# Autodesk Inventor assembly: Full Assembly
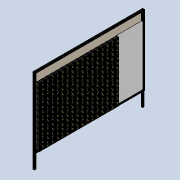
[picture p0: Inventor's stored thumbnail of the model, 180x180]
Saved by Autodesk Inventor 2022 (Build 260153000, 153)
## iProperties
Created: 2023-02-26
Part Number: Full Assembly
Document SubType Name: Assembly
Designer: byrne
Author: byrne
## Documents named in this file (7)
- C:\Users\byrne\OneDrive\Documents\Inventor\RAI\Full Assembly.iam
- C:\Users\byrne\OneDrive\Documents\Inventor\RAI\Backboard.ipt
- C:\Users\byrne\OneDrive\Documents\Inventor\RAI\56in T-Extrusion.ipt
- C:\Users\byrne\OneDrive\Documents\Inventor\RAI\70in T-Extrusion.ipt
- C:\Users\byrne\OneDrive\Documents\Inventor\RAI\Unit.iam
- C:\Users\byrne\OneDrive\Documents\Inventor\RAI\Sponsor and Ad Panel.ipt
- C:\Users\byrne\OneDrive\Documents\Inventor\RAI\98164A450_316 Stainless Steel Button Head Hex Drive Screw.ipt
## Components (202 placed, 6 different names)
1. Sponsor and Ad Panel:1 — Mate:9, Flush:11, Mate:10, Insert:1, Insert:2, Insert:3, Insert:4
2. 98164A450_316 Stainless Steel Button Head Hex Drive Screw:1 — Insert:3
3. 98164A450_316 Stainless Steel Button Head Hex Drive Screw:2 — Insert:2
4. 98164A450_316 Stainless Steel Button Head Hex Drive Screw:3 — Insert:1
5. 98164A450_316 Stainless Steel Button Head Hex Drive Screw:4 — Insert:4
6. Backboard:1 — Flush:1, Mate:1, Flush:2, Flush:4, Mate:2, Flush:5, Flush:7, Mate:3, Flush:8, Mate:6, Mate:7, Flush:10, Mate:10, Flush:12
7. 56in T-Extrusion:1 — Flush:4, Mate:2, Flush:5, Mate:8
8. 70in T-Extrusion:1 — Flush:8, Mate:6, Mate:8
9. 56in T-Extrusion:2 — Flush:1, Mate:1, Flush:2, Mate:4
10. 70in T-Extrusion:2 — Flush:7, Mate:3, Mate:4
11. Unit:1 [sub-assembly] — Mate:7, Flush:10
12. Unit:2 [sub-assembly]
13. Unit:3 [sub-assembly]
14. Unit:4 [sub-assembly]
15. Unit:5 [sub-assembly]
16. Unit:6 [sub-assembly]
17. Unit:7 [sub-assembly]
18. Unit:8 [sub-assembly]
19. Unit:9 [sub-assembly]
20. Unit:10 [sub-assembly]
21. Unit:11 [sub-assembly]
22. Unit:12 [sub-assembly]
23. Unit:13 [sub-assembly]
24. Unit:14 [sub-assembly]
25. Unit:15 [sub-assembly]
26. Unit:16 [sub-assembly]
27. Unit:17 [sub-assembly]
28. Unit:18 [sub-assembly]
29. Unit:19 [sub-assembly]
30. Unit:20 [sub-assembly]
31. Unit:21 [sub-assembly]
32. Unit:22 [sub-assembly]
33. Unit:23 [sub-assembly]
34. Unit:24 [sub-assembly]
35. Unit:25 [sub-assembly]
36. Unit:26 [sub-assembly]
37. Unit:27 [sub-assembly]
38. Unit:28 [sub-assembly]
39. Unit:29 [sub-assembly]
40. Unit:30 [sub-assembly]
41. Unit:31 [sub-assembly]
42. Unit:32 [sub-assembly]
43. Unit:33 [sub-assembly]
44. Unit:34 [sub-assembly]
45. Unit:35 [sub-assembly]
46. Unit:36 [sub-assembly]
47. Unit:37 [sub-assembly]
48. Unit:38 [sub-assembly]
49. Unit:39 [sub-assembly]
50. Unit:40 [sub-assembly]
51. Unit:41 [sub-assembly]
52. Unit:42 [sub-assembly]
53. Unit:43 [sub-assembly]
54. Unit:44 [sub-assembly]
55. Unit:45 [sub-assembly]
56. Unit:46 [sub-assembly]
57. Unit:47 [sub-assembly]
58. Unit:48 [sub-assembly]
59. Unit:49 [sub-assembly]
60. Unit:50 [sub-assembly]
61. Unit:51 [sub-assembly]
62. Unit:52 [sub-assembly]
63. Unit:53 [sub-assembly]
64. Unit:54 [sub-assembly]
65. Unit:55 [sub-assembly]
66. Unit:56 [sub-assembly]
67. Unit:57 [sub-assembly]
68. Unit:58 [sub-assembly]
69. Unit:59 [sub-assembly]
70. Unit:60 [sub-assembly]
71. Unit:61 [sub-assembly]
72. Unit:62 [sub-assembly]
73. Unit:63 [sub-assembly]
74. Unit:64 [sub-assembly]
75. Unit:65 [sub-assembly]
76. Unit:66 [sub-assembly]
77. Unit:67 [sub-assembly]
78. Unit:68 [sub-assembly]
79. Unit:69 [sub-assembly]
80. Unit:70 [sub-assembly]
81. Unit:71 [sub-assembly]
82. Unit:72 [sub-assembly]
83. Unit:73 [sub-assembly]
84. Unit:74 [sub-assembly]
85. Unit:75 [sub-assembly]
86. Unit:76 [sub-assembly]
87. Unit:77 [sub-assembly]
88. Unit:78 [sub-assembly]
89. Unit:79 [sub-assembly]
90. Unit:80 [sub-assembly]
91. Unit:81 [sub-assembly]
92. Unit:82 [sub-assembly]
93. Unit:83 [sub-assembly]
94. Unit:84 [sub-assembly]
95. Unit:85 [sub-assembly]
96. Unit:86 [sub-assembly]
97. Unit:87 [sub-assembly]
98. Unit:88 [sub-assembly]
99. Unit:89 [sub-assembly]
100. Unit:90 [sub-assembly]
101. Unit:91 [sub-assembly]
102. Unit:92 [sub-assembly]
103. Unit:93 [sub-assembly]
104. Unit:94 [sub-assembly]
105. Unit:95 [sub-assembly]
106. Unit:96 [sub-assembly]
107. Unit:97 [sub-assembly]
108. Unit:98 [sub-assembly]
109. Unit:99 [sub-assembly]
110. Unit:100 [sub-assembly]
111. Unit:101 [sub-assembly]
112. Unit:102 [sub-assembly]
113. Unit:103 [sub-assembly]
114. Unit:104 [sub-assembly]
115. Unit:105 [sub-assembly]
116. Unit:106 [sub-assembly]
117. Unit:107 [sub-assembly]
118. Unit:108 [sub-assembly]
119. Unit:109 [sub-assembly]
120. Unit:110 [sub-assembly]
121. Unit:111 [sub-assembly]
122. Unit:112 [sub-assembly]
123. Unit:113 [sub-assembly]
124. Unit:114 [sub-assembly]
125. Unit:115 [sub-assembly]
126. Unit:116 [sub-assembly]
127. Unit:117 [sub-assembly]
128. Unit:118 [sub-assembly]
129. Unit:119 [sub-assembly]
130. Unit:120 [sub-assembly]
131. Unit:121 [sub-assembly]
132. Unit:122 [sub-assembly]
133. Unit:123 [sub-assembly]
134. Unit:124 [sub-assembly]
135. Unit:125 [sub-assembly]
136. Unit:126 [sub-assembly]
137. Unit:127 [sub-assembly]
138. Unit:128 [sub-assembly]
139. Unit:129 [sub-assembly]
140. Unit:130 [sub-assembly]
141. Unit:131 [sub-assembly]
142. Unit:132 [sub-assembly]
143. Unit:133 [sub-assembly]
144. Unit:134 [sub-assembly]
145. Unit:135 [sub-assembly]
146. Unit:136 [sub-assembly]
147. Unit:137 [sub-assembly]
148. Unit:138 [sub-assembly]
149. Unit:139 [sub-assembly]
150. Unit:140 [sub-assembly]
151. Unit:141 [sub-assembly]
152. Unit:142 [sub-assembly]
153. Unit:143 [sub-assembly]
154. Unit:144 [sub-assembly]
155. Unit:145 [sub-assembly]
156. Unit:146 [sub-assembly]
157. Unit:147 [sub-assembly]
158. Unit:148 [sub-assembly]
159. Unit:149 [sub-assembly]
160. Unit:150 [sub-assembly]
161. Unit:151 [sub-assembly]
162. Unit:152 [sub-assembly]
163. Unit:153 [sub-assembly]
164. Unit:154 [sub-assembly]
165. Unit:155 [sub-assembly]
166. Unit:156 [sub-assembly]
167. Unit:157 [sub-assembly]
168. Unit:158 [sub-assembly]
169. Unit:159 [sub-assembly]
170. Unit:160 [sub-assembly]
171. Unit:161 [sub-assembly]
172. Unit:162 [sub-assembly]
173. Unit:163 [sub-assembly]
174. Unit:164 [sub-assembly]
175. Unit:165 [sub-assembly]
176. Unit:166 [sub-assembly]
177. Unit:167 [sub-assembly]
178. Unit:168 [sub-assembly]
179. Unit:169 [sub-assembly]
180. Unit:170 [sub-assembly]
181. Unit:171 [sub-assembly]
182. Unit:172 [sub-assembly]
183. Unit:173 [sub-assembly]
184. Unit:174 [sub-assembly]
185. Unit:175 [sub-assembly]
186. Unit:176 [sub-assembly]
187. Unit:177 [sub-assembly] — Flush:12
188. Unit:178 [sub-assembly]
189. Unit:179 [sub-assembly]
190. Unit:180 [sub-assembly]
191. Unit:181 [sub-assembly]
192. Unit:182 [sub-assembly]
193. Unit:183 [sub-assembly]
194. Unit:184 [sub-assembly]
195. Unit:185 [sub-assembly]
196. Unit:186 [sub-assembly]
197. Unit:187 [sub-assembly]
198. Unit:188 [sub-assembly]
199. Unit:189 [sub-assembly]
200. Unit:190 [sub-assembly]
201. Unit:191 [sub-assembly]
202. Unit:192 [sub-assembly] — Mate:9, Flush:11
## Component patterns: (192 elements, first: Unit:1)
## Relationships (22: Flush 9, Mate 9, Insert 4)
- Flush:1: Backboard:1 ↔ 56in T-Extrusion:2
- Mate:1: Backboard:1 ↔ 56in T-Extrusion:2
- Flush:2: Backboard:1 ↔ 56in T-Extrusion:2
- Flush:4: Backboard:1 ↔ 56in T-Extrusion:1
- Mate:2: Backboard:1 ↔ 56in T-Extrusion:1
- Flush:5: Backboard:1 ↔ 56in T-Extrusion:1
- Flush:7: Backboard:1 ↔ 70in T-Extrusion:2
- Mate:3: Backboard:1 ↔ 70in T-Extrusion:2
- Mate:4: 56in T-Extrusion:2 ↔ 70in T-Extrusion:2
- Flush:8: Backboard:1 ↔ 70in T-Extrusion:1
- Mate:6: Backboard:1 ↔ 70in T-Extrusion:1
- Mate:7: Backboard:1 ↔ Unit:1
- Flush:10 (44.45 mm): Backboard:1 ↔ Unit:1
- Mate:8: 56in T-Extrusion:1 ↔ 70in T-Extrusion:1
- Mate:9 (6.35 mm): Sponsor and Ad Panel:1 ↔ Unit:192
- Flush:11: Sponsor and Ad Panel:1 ↔ Unit:192
- Mate:10: Sponsor and Ad Panel:1 ↔ Backboard:1
- Flush:12 (44.45 mm): Backboard:1 ↔ Unit:177
- Insert:1: Sponsor and Ad Panel:1 ↔ 98164A450_316 Stainless Steel Button Head Hex Drive Screw:3
- Insert:2: Sponsor and Ad Panel:1 ↔ 98164A450_316 Stainless Steel Button Head Hex Drive Screw:2
- Insert:3: Sponsor and Ad Panel:1 ↔ 98164A450_316 Stainless Steel Button Head Hex Drive Screw:1
- Insert:4: Sponsor and Ad Panel:1 ↔ 98164A450_316 Stainless Steel Button Head Hex Drive Screw:4
